# Autodesk Inventor assembly: !Intake
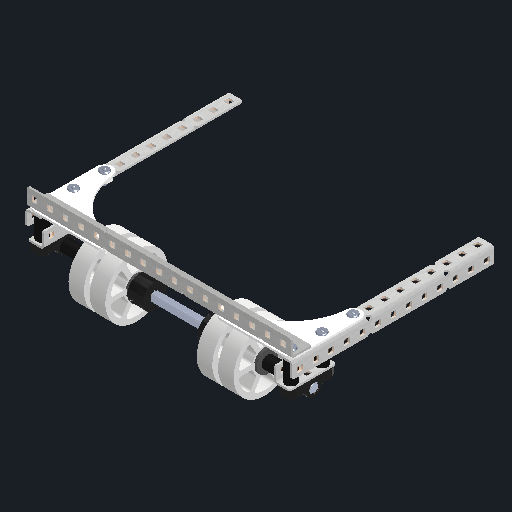
[picture p0: Inventor's stored thumbnail of the model, 512x512]
Saved by Autodesk Inventor 2025 (Build 290162000, 162)
## iProperties
Created: 2024-10-21
Part Number: !Intake
Document SubType Name: Assembly
Designer: averey
Author: averey
## Documents named in this file (4)
- D:\VEX\High Stakes\CAD\V2\Intake\Floating Stage\!Floating Stage.iam
- !Floating Stage.iam
- D:\VEX\High Stakes\CAD\V2\Intake\Floating Stage\Structure.iam
- D:\VEX\High Stakes\CAD\V2\Intake\Floating Stage\Pre-roller.iam
## Components (2 placed, 2 different names)
1. Structure:1 [sub-assembly] — Insert:1
2. Pre-roller:1 [sub-assembly] — Insert:1
## Relationships (1: Insert 1)
- Insert:1: Structure:1 ↔ Pre-roller:1
